# Autodesk Inventor assembly: SDA32x25(0)+()
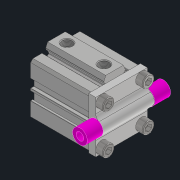
[picture p0: Inventor's stored thumbnail of the model, 180x180]
Saved by Autodesk Inventor 2022 (Build 260153000, 153)
## iProperties
Category: PARTsolutions
Company: AIRTAC
Created: 2022-09-20
Part Number: SDA32x25(0)+()
Catalog Web Link: www.cadenas.de
Description: SDA SSA STA-Compact Cylinder
Vendor: AIRTAC
Document SubType Name: Assembly
Designer: psAdmin
Manufacturer: AIRTAC
Mass: 67.1382 g
Surface Area: 299.521 cm^2
Volume: 67.1382 cm^3
Density: 1 g/cm^3
PSOL_IDENT_0: {$CADENAS_DATA/23d-libs/airtac/pneumatic_equipment/cylinders/compact_cylinder/sda_series/sda_ssa_sta
PSOL_IDENT_1: _asmtab.prj},258 {VTYP=3D},{STYP=ASSTAB},{NB=SDA32x25(0)+()},{LINA=SDA32x25(0)+()},{NN=SDA SSA STA},
PSOL_IDENT_2: {DATE=21.07.2022 03:23:18},{GEOMDATE=16.11.2020 05:39:27},{VERSION=},{LINEID=50},{WBVAR=TYPE,STROKE,
PSOL_IDENT_3: MAGNET,RTYPE,THREAD,POS,SENSORSWITCH,SENSORNUMBER},{WBNUMERIC=STROKE,POS}  {NB=SDA32x25(0)+()},{LINA=
PSOL_IDENT_4: SDA32x25(0)+()},{KT=DUMMY},{MODEL=SDA32x25},{TYPE=SDA},{BORE=32},{STROKE=25},{MAGNET=},{RTYPE=},{THR
PSOL_IDENT_5: EAD=},{POS=0},{SENSORSWITCH=},{SENSORNUMBER=},{INFO=PDF Catalogues},{ST1=5,10,15,20,25,30,35,40,45,5
PSOL_IDENT_6: 0,55,60,65,70,75,80,85,90,100,110,120,130,[5:130]},{ORDER=SDA32x25},{A=31.5},{B1=7},{B2=-},{C=24.5},
PSOL_IDENT_7: {D=50},{E=12},{F=4},{G=3.0},{H=-},{I=-},{J=-},{K1=M6x1.0},{K2=-},{L=22.0},{M=3},{N1=9.0},{N2=9.0},{O=
PSOL_IDENT_8: 1/8\"},{P1=4.6},{P2=M6x1.0},{P3=16},{P4=5.5},{P5=8.2},{R=6},{S=44},{T1=34.0},{T2=-},{U=2.0},{V=12},{
PSOL_IDENT_9: W=10},{X=18.3},{Y=15},{TYPE1='SDA', 'SDA Type', 'SSA', 'SSA Type', 'STA', 'STA Type'},{PPATH=assembl
PSOL_IDENT_10: ies/sda_ssa_sta_asmtpl.prj},{PRA=2},{TH1='', 'PT', 'T', 'NPT', 'G', 'G'},{SW='','N/A'},{SN='','N/A'}
PSOL_IDENT_11: ,{RTH=},{SWH=},{CNSTYPECODE=SDA32x25},{MSMNO=SDA-32X25}
NB: SDA32x25(0)+()
NN: SDA SSA STA
NT: Compact Cylinder
NBSYN: $TYPE.$BORE.x$STROKE.$MAGNET.$RTH.$THREAD.($POS.)+($SWH.$SENSORNUMBER.)
LINA: SDA32x25(0)+()
CATALOG: AirTAC
MODEL: SDA32x25
TYPE: SDA Type
BORE: 32
STROKE: 25
MAGNET: Without magnet
RTYPE: Female thread
THREAD: PT
POS: 0
SENSORSWITCH: N/A
SENSORNUMBER: N/A
A: 31.5
B1: 7
B2: -
C: 24.5
D: 50
E: 12
F: 4
G: 3
H: -
I: -
J: -
K1: M6x1.0
K2: -
L: 22
M: 3
N1: 9
N2: 9
O: 1/8"
P1: 4.6
P2: M6x1.0
P3: 16
P4: 5.5
P5: 8.2
R: 6
S: 44
T1: 34
T2: -
V: 12
W: 10
X: 18.3
Y: 15
SUPPLIER: AIRTAC
ARTICLENO: SDA32x25(0)+()
BOMINFO: SDA32x25(0)+()
CREATOR: CADENAS GmbH
Title: SDA32x25(0)+()
Author: Cadenas PARTsolutions
Comments: Compact Cylinder
## Documents named in this file (7)
- C:\Users\robpl\OneDrive\Documents\Inventor\WASP\Wasp\AIS2022\SDA32x25(0)+().iam
- C:\Users\robpl\OneDrive\Documents\Inventor\WASP\Wasp\AIS2022\SDA-32x2525_b.ipt
- C:\Users\robpl\OneDrive\Documents\Inventor\WASP\Wasp\AIS2022\SDA-32x2525_r.ipt
- C:\Users\robpl\OneDrive\Documents\Inventor\WASP\Wasp\Piston Mount.ipt
- C:\Users\robpl\OneDrive\Documents\Inventor\WASP\Wasp\16mm M6 Spacer.ipt
- C:\Users\robpl\OneDrive\Documents\Inventor\Content Center Files\R2022\en-US\ISO 4762(2)\ISO 4762 - M6 x 16ISO.ipt
- C:\Users\robpl\OneDrive\Documents\Inventor\Content Center Files\R2022\en-US\ISO 4762(2)\ISO 4762 - M6 x 20ISO.ipt
## Components (13 placed, 6 different names)
1. SDA-32x2525_b:1 — for_dummy_Z@1 <-> for_body_Z@2, for_dummy_YZ@1 <-> for_body_YZ@2, Flush:1, Mate:2, Mate:3, Mate:4
2. SDA-32x2525_r:1 — for_dummy_Z@1 <-> for_body_Z@2, for_dummy_YZ@1 <-> for_body_YZ@2, Flush:1
3. Piston Mount:1 — Mate:2, Mate:3, Mate:4, Mate:6, Mate:7, Mate:8, Mate:9, Mate:10, Mate:11, Mate:12, Mate:13, Mate:14, Mate:15, Mate:16, Mate:17, Mate:18, Mate:19, Mate:20, Mate:21, Mate:22, Mate:23, Mate:24
4. 16mm M6 Spacer:1 — Mate:5, Mate:6, Mate:7
5. 16mm M6 Spacer:2 — Mate:5, Mate:8
6. ISO 4762 M6 x 16:1 — Mate:9, Mate:10
7. ISO 4762 M6 x 16:2 — Mate:11, Mate:12
8. ISO 4762 M6 x 16:3 — Mate:13, Mate:14
9. ISO 4762 M6 x 16:4 — Mate:15, Mate:16
10. ISO 4762 M6 x 20:1 — Mate:17, Mate:18
11. ISO 4762 M6 x 16:6 — Mate:19, Mate:20
12. ISO 4762 M6 x 16:7 — Mate:21, Mate:22
13. ISO 4762 M6 x 16:8 — Mate:23, Mate:24
## Relationships (26: Mate 24, Angle 1, Flush 1)
- for_dummy_Z@1 <-> for_body_Z@2 [Mate]: SDA-32x2525_b:1 ↔ SDA-32x2525_r:1
- for_dummy_YZ@1 <-> for_body_YZ@2 [Angle] (90 deg): SDA-32x2525_b:1 ↔ SDA-32x2525_r:1
- Flush:1 (4 mm): SDA-32x2525_b:1 ↔ SDA-32x2525_r:1
- Mate:2: SDA-32x2525_b:1 ↔ Piston Mount:1
- Mate:3: SDA-32x2525_b:1 ↔ Piston Mount:1
- Mate:4: SDA-32x2525_b:1 ↔ Piston Mount:1
- Mate:5: 16mm M6 Spacer:1 ↔ 16mm M6 Spacer:2
- Mate:6: Piston Mount:1 ↔ 16mm M6 Spacer:1
- Mate:7: Piston Mount:1 ↔ 16mm M6 Spacer:1
- Mate:8: Piston Mount:1 ↔ 16mm M6 Spacer:2
- Mate:9: Piston Mount:1 ↔ ISO 4762 M6 x 16:1
- Mate:10: Piston Mount:1 ↔ ISO 4762 M6 x 16:1
- Mate:11: Piston Mount:1 ↔ ISO 4762 M6 x 16:2
- Mate:12: Piston Mount:1 ↔ ISO 4762 M6 x 16:2
- Mate:13: Piston Mount:1 ↔ ISO 4762 M6 x 16:3
- Mate:14: Piston Mount:1 ↔ ISO 4762 M6 x 16:3
- Mate:15: Piston Mount:1 ↔ ISO 4762 M6 x 16:4
- Mate:16: Piston Mount:1 ↔ ISO 4762 M6 x 16:4
- Mate:17: Piston Mount:1 ↔ ISO 4762 M6 x 20:1
- Mate:18: Piston Mount:1 ↔ ISO 4762 M6 x 20:1
- Mate:19: Piston Mount:1 ↔ ISO 4762 M6 x 16:6
- Mate:20: Piston Mount:1 ↔ ISO 4762 M6 x 16:6
- Mate:21: Piston Mount:1 ↔ ISO 4762 M6 x 16:7
- Mate:22: Piston Mount:1 ↔ ISO 4762 M6 x 16:7
- Mate:23: Piston Mount:1 ↔ ISO 4762 M6 x 16:8
- Mate:24: Piston Mount:1 ↔ ISO 4762 M6 x 16:8
